# Autodesk Inventor assembly: table
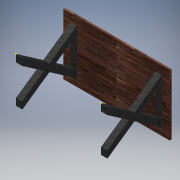
[picture p0: Inventor's stored thumbnail of the model, 180x180]
Saved by Autodesk Inventor 2019 (Build 230136000, 136)
## iProperties
Created: 2019-07-26
Part Number: table
Document SubType Name: Assembly
Designer: Alex
Author: Alex
## Documents named in this file (3)
- P:\Alex\Git\3d_models\dining_table\x-legs\table.iam
- P:\Alex\Git\3d_models\dining_table\x-legs\leg.ipt
- P:\Alex\Git\3d_models\dining_table\x-legs\tabletop.ipt
## Components (3 placed, 2 different names)
1. leg:1 — Mate:1, Angle:1, Flush:2, Flush:3, Flush:4
2. leg:2 — Mate:2, Flush:1, Flush:4
3. tabletop:1 — Mate:1, Mate:2, Angle:1, Flush:1, Flush:2, Flush:3
## Relationships (7: Flush 4, Mate 2, Angle 1)
- Mate:1: leg:1 ↔ tabletop:1
- Mate:2: leg:2 ↔ tabletop:1
- Angle:1 (0 deg): leg:1 ↔ tabletop:1
- Flush:1 (100 mm): leg:2 ↔ tabletop:1
- Flush:2 (100 mm): leg:1 ↔ tabletop:1
- Flush:3 (-100 mm): leg:1 ↔ tabletop:1
- Flush:4: leg:1 ↔ leg:2
